# Autodesk Inventor assembly: Assembly1
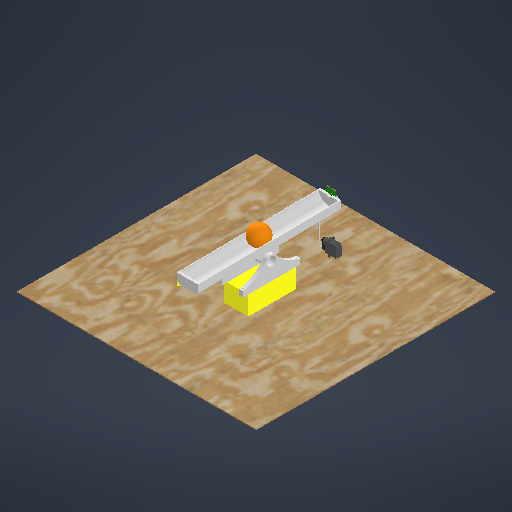
[picture p0: Inventor's stored thumbnail of the model, 512x512]
Saved by Autodesk Inventor 2026.2 (Build 302298000, 298)
## iProperties
Created: 2025-12-09
Part Number: Assembly1
Document SubType Name: Assembly
Designer: janek
Author: janek
## iProperties of the stored document MG90S Micro Servo Motor.iam
Created: 2025-06-12
Part Number: MG90S Micro Servo Motor
Document SubType Name: Assembly
Designer: janek
Sending System: Autodesk Translation Framework v14.10.0.0
Preprocessor: ST-DEVELOPER v20.1
Title: MG90S Micro Servo Motor.step
## iProperties of the stored document Horn.ipt
Created: 2025-12-09
Part Number: Horn
Material: Steel
Document SubType Name: Modeling
Designer: janek
Density: 7.85 g/cm^3
Appearance: Default
Author: janek
## iProperties of the stored document Body.ipt
Created: 2025-12-09
Part Number: Body
Material: Steel
Document SubType Name: Modeling
Designer: janek
Density: 7.85 g/cm^3
Appearance: Default
Author: janek
## iProperties of the stored document Screw.ipt
Created: 2025-12-09
Part Number: Screw
Material: Steel
Document SubType Name: Modeling
Designer: janek
Density: 7.85 g/cm^3
Appearance: Default
Author: janek
## iProperties of the stored document Shaft.ipt
Created: 2025-12-09
Part Number: Shaft
Material: Steel
Document SubType Name: Modeling
Designer: janek
Density: 7.85 g/cm^3
Appearance: Default
Author: janek
## Documents named in this file (15)
- C:\Users\janek\Documents\stmprojekt\STM_PROJEKT_ZALICZENIOWY\inventormodel\assembly\Assembly1.iam
- C:\Users\janek\Documents\stmprojekt\STM_PROJEKT_ZALICZENIOWY\inventormodel\ramp\profilrampa.ipt
- C:\Users\janek\Documents\stmprojekt\STM_PROJEKT_ZALICZENIOWY\inventormodel\ramp\pingpongball.ipt
- C:\Users\janek\Documents\stmprojekt\STM_PROJEKT_ZALICZENIOWY\inventormodel\Grove - Time of Flight Distance Sensor (VL53L0X)\202002000_PCBA;Grove - Time of Flight Distance Sensor (VL53L0X)_原理图\Grove-Time-of-Flight-Distance-SensorVL53L0X\Grove.iam
- C:\Users\janek\Documents\stmprojekt\STM_PROJEKT_ZALICZENIOWY\inventormodel\ramp\podstawa.ipt
- C:\Users\janek\Documents\stmprojekt\STM_PROJEKT_ZALICZENIOWY\inventormodel\ramp\drut.ipt
- C:\Users\janek\Documents\stmprojekt\STM_PROJEKT_ZALICZENIOWY\inventormodel\ramp\placeholder.ipt
- C:\Users\janek\Documents\stmprojekt\STM_PROJEKT_ZALICZENIOWY\inventormodel\ramp\podloga.ipt
- **C:\Users\janek\Documents\stmprojekt\STM_PROJEKT_ZALICZENIOWY\inventormodel\assembly\Assembly1.iam*LocalDocs*xAaaaandaAaaaaaaaAaaaakviPe*MG90S Micro Servo Motor.iam
- **C:\Users\janek\Documents\stmprojectinventor\assembly\Assembly1.iam*LocalDocs*xAaaaandaAaaaaaaaAaaaakviPe*MG90S Micro Servo Motor.iam
- **C:\Users\janek\Documents\stmprojectinventor\assembly\Assembly1.iam*LocalDocs*xAaaaqtaaAaaaaaaaAaaaqgqqWf*Body.ipt
- **C:\Users\janek\Documents\stmprojectinventor\assembly\Assembly1.iam*LocalDocs*xAaaaqvcaAaaaaaaaAaaaqwh2Oc*Shaft.ipt
- **C:\Users\janek\Documents\stmprojectinventor\assembly\Assembly1.iam*LocalDocs*xAaaaahbaAaaaaaaaAaaaq03xXd*Horn.ipt
- **C:\Users\janek\Documents\stmprojectinventor\assembly\Assembly1.iam*LocalDocs*xAaaaawaaAaaaaaaaAaaaqxdeGa*Screw.ipt
- C:\Users\janek\Documents\stmprojekt\STM_PROJEKT_ZALICZENIOWY\inventormodel\mg90s-micro-servo-motor-1\MG90S Micro Servo Motor\MG90S Micro Servo Motor.step
## Components (9 placed, 8 different names)
1. profilrampa:1 — Rigid:1, Mate:1, Mate:2, Mate:3, Mate:4, Mate:5, Mate:6, Mate:7, Mate:8, Flush:1
2. pingpongball:1 — Rigid:1
3. Grove:1 [sub-assembly] — Mate:1, Mate:2, Mate:3
4. podstawa:1 — Mate:4, Mate:5, Flush:2, Mate:11, Mate:12
5. podstawa:2 — Mate:6, Mate:7, Mate:10
6. drut:1 — Mate:8, Flush:1, Mate:14
7. placeholder:1 — Mate:10, Flush:2, Mate:11, Mate:12, Mate:13
8. podloga:1 — Mate:13
9. MG90S Micro Servo Motor:1 [sub-assembly] — Mate:14
## Relationships (16: Mate 13, Flush 2, WeldJoint 1)
- Rigid:1 [WeldJoint]: profilrampa:1 ↔ pingpongball:1
- Mate:1: profilrampa:1 ↔ Grove:1
- Mate:2: profilrampa:1 ↔ Grove:1
- Mate:3: profilrampa:1 ↔ Grove:1
- Mate:4: profilrampa:1 ↔ podstawa:1
- Mate:5: profilrampa:1 ↔ podstawa:1
- Mate:6: profilrampa:1 ↔ podstawa:2
- Mate:7: profilrampa:1 ↔ podstawa:2
- Mate:8: profilrampa:1 ↔ drut:1
- Flush:1 (-2 mm): profilrampa:1 ↔ drut:1
- Mate:10: podstawa:2 ↔ placeholder:1
- Flush:2: podstawa:1 ↔ placeholder:1
- Mate:11: podstawa:1 ↔ placeholder:1
- Mate:12: podstawa:1 ↔ placeholder:1
- Mate:13: placeholder:1 ↔ podloga:1
- Mate:14: drut:1 ↔ MG90S Micro Servo Motor:1
